# Autodesk Inventor assembly: 2XL-430montado
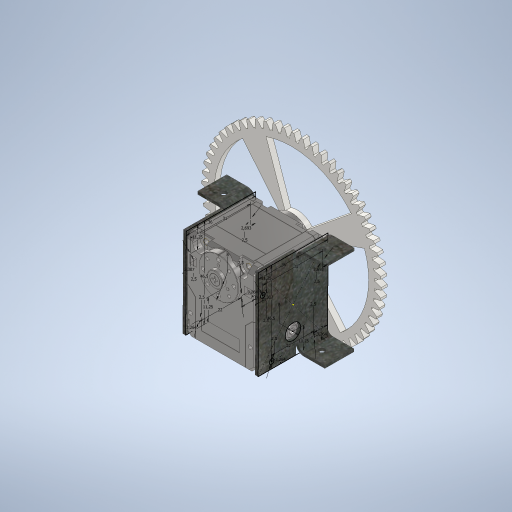
[picture p0: Inventor's stored thumbnail of the model, 512x512]
Saved by Autodesk Inventor 2023 (Build 270158000, 158)
## iProperties
Created: 2019-05-16
Part Number: 2XL-430montado
Document SubType Name: Assembly
Designer: hiago.sodre
Sending System: CREO PARAMETRIC BY PTC INC, 2018260
Preprocessor: CREO PARAMETRIC BY PTC INC, 2018260
Title: DC14_A01_REF_ASM
Author: eum
Revision Number: 5LAST_VERSION
## Documents named in this file (12)
- C:\Users\hiago.sodre\Downloads\MODELO2XL-430\Model_2XL430-W250-T\2XL-430montado.iam
- C:\Users\hiago.sodre\Downloads\MODELO2XL-430\Model_2XL430-W250-T\DC14_A01_REF.ipt
- C:\Users\hiago.sodre\Downloads\MODELO2XL-430\Model_2XL430-W250-T\S3B-EH.ipt
- C:\Users\hiago.sodre\Downloads\MODELO2XL-430\Model_2XL430-W250-T\EHR-3.ipt
- C:\Users\hiago.sodre\Downloads\MODELO2XL-430\Model_2XL430-W250-T\PHS_M2X33_TAP_K.ipt
- C:\Users\hiago.sodre\Downloads\MODELO2XL-430\Model_2XL430-W250-T\DC14_A01_INSERT_2.ipt
- C:\Users\hiago.sodre\Downloads\MODELO2XL-430\Model_2XL430-W250-T\DC14_A01_INSERT_1.ipt
- C:\Users\hiago.sodre\Downloads\MODELO2XL-430\Model_2XL430-W250-T\DC11_A01_HORN_REF_ASM.iam
- C:\Users\hiago.sodre\Downloads\MODELO2XL-430\Model_2XL430-W250-T\DC11_A01_IDLER_REF_ASM.iam
- C:\Users\hiago.sodre\Downloads\MODELO2XL-430\Model_2XL430-W250-T\Engrenaje.iam
- C:\Users\hiago.sodre\Downloads\MODELO2XL-430\Model_2XL430-W250-T\Soporte_Motor_2XL_D_chapa.ipt
- C:\Users\hiago.sodre\Downloads\MODELO2XL-430\Model_2XL430-W250-T\Soporte_Motor_2XL_E_chapa.ipt
## Components (24 placed, 24 different names)
1. 68 — Rotativa:2, De rotación:3, De rotación:4
2. 69
3. 70
4. 71
5. 72
6. 73
7. 74
8. 75
9. 76
10. 77
11. 78
12. 79
13. 80
14. 81
15. 82
16. 83
17. 84
18. 85
19. 86
20. 90 [sub-assembly]
21. 95 [sub-assembly] — Rotativa:1, Rotativa:2
22. Engrenaje:1 [sub-assembly] — Rotativa:1
23. Soporte_Motor_2XL_D_chapa:1 — De rotación:4
24. Soporte_Motor_2XL_E_chapa:1 — De rotación:3
## Relationships (4: RevoluteJoint 4)
- Rotativa:1 [RevoluteJoint]: 95 ↔ Engrenaje:1
- Rotativa:2 [RevoluteJoint]: 68 ↔ 95
- De rotación:3 [RevoluteJoint]: 68 ↔ Soporte_Motor_2XL_E_chapa:1
- De rotación:4 [RevoluteJoint]: 68 ↔ Soporte_Motor_2XL_D_chapa:1
